# Autodesk Inventor assembly: Eye Bolt and Nut
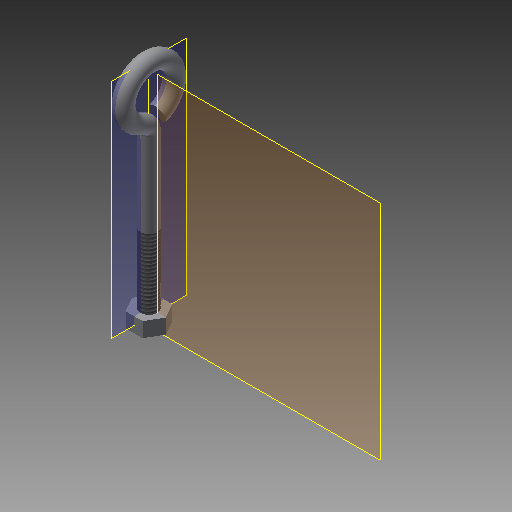
[picture p0: Inventor's stored thumbnail of the model, 512x512]
Saved by Autodesk Inventor 2018.2 (Build 222227000, 227)
## iProperties
Created: 2018-03-13
Part Number: Eye Bolt and Nut
Document SubType Name: Assembly
Designer: owner
Author: owner
## Documents named in this file (3)
- Z:\The Pickle\Final Carts\Eye Bolt and Nut.iam
- Z:\The Pickle\Final Carts\Locking Mech\Eyebolt Nut.ipt
- Z:\The Pickle\Final Carts\Locking Mech\Eyebolt.ipt
## Components (2 placed, 2 different names)
1. Eyebolt Nut:1 — Insert:1
2. Eyebolt:1 — Insert:1, Angle:1, Mate:1, Mate:2
## Relationships (6: Mate 3, Angle 2, Insert 1)
- Insert:1: Eyebolt Nut:1 ↔ Eyebolt:1
- Angle:1 (0 deg): Eyebolt:1
- Mate:1: Eyebolt:1
- Mate:2: Eyebolt:1
- Mate:3
- Angle:2 (90 deg)
